# Autodesk Inventor assembly: единое крепление
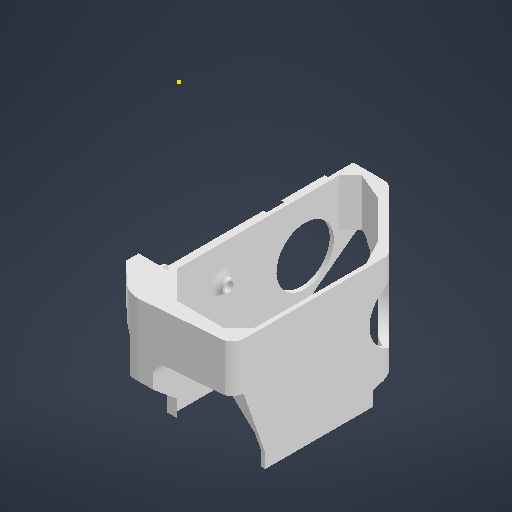
[picture p0: Inventor's stored thumbnail of the model, 512x512]
Saved by Autodesk Inventor 2025 (Build 290162000, 162)
## iProperties
Created: 2024-09-25
Part Number: единое крепление
Document SubType Name: Assembly
Designer: GameHD
Author: GameHD
## Documents named in this file (3)
- C:\Users\GameHD\Desktop\что-то нужное\Phantom16950\единое крепление.iam
- C:\Users\GameHD\Desktop\что-то нужное\Phantom16950\крепл для колёс встав часть.ipt
- C:\Users\GameHD\Desktop\что-то нужное\Phantom16950\крепл для колёс.ipt
## Components (2 placed, 2 different names)
1. крепл для колёс встав часть:1 — Совмещение:1, Заподлицо:1, Заподлицо:2
2. крепл для колёс:1 — Совмещение:1, Заподлицо:1, Заподлицо:2
## Relationships (3: Flush 2, Mate 1)
- Совмещение:1 [Mate]: крепл для колёс встав часть:1 ↔ крепл для колёс:1
- Заподлицо:1 [Flush]: крепл для колёс встав часть:1 ↔ крепл для колёс:1
- Заподлицо:2 [Flush]: крепл для колёс встав часть:1 ↔ крепл для колёс:1
